# Autodesk Inventor assembly: prostkatna waska wysoka lacznik v2
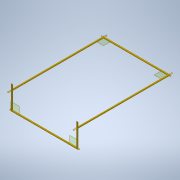
[picture p0: Inventor's stored thumbnail of the model, 180x180]
Saved by Autodesk Inventor 2021 (Build 250183000, 183)
## iProperties
Created: 2024-04-18
Part Number: prostkatna waska wysoka lacznik v2
Document SubType Name: Assembly
Designer: Michal
Author: Michal
## Documents named in this file (5)
- C:\Users\Michal\Documents\GitHub\PNW_PhotoBoothFrame_3D\prostkatna waska wysoka lacznik v2.iam
- C:\Users\Michal\Documents\GitHub\PNW_PhotoBoothFrame_3D\Naroznik v2.iam
- C:\Users\Michal\Documents\GitHub\PNW_PhotoBoothFrame_3D\Przedluzka L2400.ipt
- C:\Users\Michal\Documents\GitHub\PNW_PhotoBoothFrame_3D\Przedluzka L1680.ipt
- C:\Users\Michal\Documents\GitHub\PNW_PhotoBoothFrame_3D\Stopa v4.iam
## Components (10 placed, 4 different names)
1. Naroznik v2:1 [sub-assembly] — Mate:11
2. Przedluzka L2400:1 — Mate:11, Mate:14, Flush:5, Mate:15
3. Przedluzka L1680:1 — Mate:13
4. Naroznik v2:2 [sub-assembly] — Mate:12, Mate:13
5. Przedluzka L2400:2 — Mate:12, Flush:18, Mate:18, Mate:19
6. Stopa v4:1 [sub-assembly] — Mate:14, Flush:5, Mate:15, Flush:6, Flush:17, Mate:17
7. Naroznik v2:3 [sub-assembly] — Flush:6, Flush:17, Mate:17
8. Stopa v4:2 [sub-assembly] — Flush:18, Mate:18, Mate:19, Flush:19, Flush:20, Mate:20
9. Naroznik v2:4 [sub-assembly] — Flush:19, Flush:20, Mate:20, Mate:21, Mate:22, Mate:23
10. Przedluzka L1680:2 — Mate:21, Mate:22, Mate:23
## Relationships (30: Mate 22, Flush 8)
- [Mate]: Naroznik v2:1 ↔ Przedluzka L2400:1
- [Mate]: Naroznik v2:1 ↔ Przedluzka L2400:1
- [Flush]: Naroznik v2:1 ↔ Przedluzka L1680:1
- [Mate]: Naroznik v2:1 ↔ Przedluzka L1680:1
- [Mate]: Naroznik v2:1 ↔ Przedluzka L1680:1
- [Mate]: Naroznik v2:2 ↔ Przedluzka L2400:2
- [Mate]: Naroznik v2:2 ↔ Przedluzka L2400:2
- [Mate]: Naroznik v2:2 ↔ Przedluzka L2400:2
- [Flush]: Przedluzka L1680:1 ↔ Przedluzka L2400:2
- [Mate]: Przedluzka L1680:1 ↔ Naroznik v2:2
- [Mate]: Przedluzka L1680:1 ↔ Naroznik v2:2
- [Mate]: Naroznik v2:1 ↔ Przedluzka L2400:1
- Mate:11: Naroznik v2:1 ↔ Przedluzka L2400:1
- Mate:12: Naroznik v2:2 ↔ Przedluzka L2400:2
- Mate:13: Przedluzka L1680:1 ↔ Naroznik v2:2
- Mate:14: Przedluzka L2400:1 ↔ Stopa v4:1
- Flush:5: Przedluzka L2400:1 ↔ Stopa v4:1
- Mate:15: Przedluzka L2400:1 ↔ Stopa v4:1
- Flush:6: Stopa v4:1 ↔ Naroznik v2:3
- Flush:17: Stopa v4:1 ↔ Naroznik v2:3
- Mate:17: Stopa v4:1 ↔ Naroznik v2:3
- Flush:18: Przedluzka L2400:2 ↔ Stopa v4:2
- Mate:18: Przedluzka L2400:2 ↔ Stopa v4:2
- Mate:19: Przedluzka L2400:2 ↔ Stopa v4:2
- Flush:19: Stopa v4:2 ↔ Naroznik v2:4
- Flush:20: Stopa v4:2 ↔ Naroznik v2:4
- Mate:20: Stopa v4:2 ↔ Naroznik v2:4
- Mate:21: Naroznik v2:4 ↔ Przedluzka L1680:2
- Mate:22: Naroznik v2:4 ↔ Przedluzka L1680:2
- Mate:23: Naroznik v2:4 ↔ Przedluzka L1680:2
